# Autodesk Inventor assembly: FumeBOT
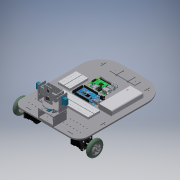
[picture p0: Inventor's stored thumbnail of the model, 180x180]
Saved by Autodesk Inventor 2018 (Build 220112000, 112)
## iProperties
Created: 2018-05-02
Part Number: FumeBOT
Document SubType Name: Assembly
Designer: Ajith Thomas
Author: Ajith Thomas
## Documents named in this file (11)
- C:\Users\Ajith Thomas\Dropbox\Gas_Sensing_Robot\FumeBot-Design\FumeBOT - with pan and tilt.iam
- C:\Users\Ajith Thomas\Dropbox\Gas_Sensing_Robot\FumeBot-Design\Base.ipt
- C:\Users\Ajith Thomas\Dropbox\Gas_Sensing_Robot\FumeBot-Design\Sensors and Boards\Raspberry Pi 3B.ipt
- C:\Users\Ajith Thomas\Dropbox\Gas_Sensing_Robot\FumeBot-Design\Sensors and Boards\Arduino MEGA 2560 R3\Arduino MEGA 2560 R3.iam
- C:\Users\Ajith Thomas\Dropbox\Gas_Sensing_Robot\FumeBot-Design\Large Bread Board.ipt
- C:\Users\Ajith Thomas\Dropbox\Gas_Sensing_Robot\FumeBot-Design\Small Bread Board.ipt
- C:\Users\Ajith Thomas\Dropbox\Gas_Sensing_Robot\FumeBot-Design\Battery.ipt
- C:\Users\Ajith Thomas\Dropbox\Gas_Sensing_Robot\FumeBot-Design\Stepper with bracket.iam
- C:\Users\Ajith Thomas\Dropbox\Gas_Sensing_Robot\FumeBot-Design\Wheel height spacers.ipt
- C:\Users\Ajith Thomas\Dropbox\Gas_Sensing_Robot\FumeBot-Design\Mecanum with supports.iam
- C:\Users\Ajith Thomas\Dropbox\Gas_Sensing_Robot\FumeBot-Design\Pan and tilt assembly\Camera pan and tilt assembly.iam
## Components (12 placed, 10 different names)
1. Base:1 — Mate:1, Mate:2, Flush:1, Flush:2, Flush:3, Flush:4, Mate:4, Mate:5, Mate:6, Flush:6, Flush:7, Mate:7, Mate:8, Mate:9, Mate:10, Mate:11, Mate:12, Flush:8, Mate:13
2. Raspberry Pi 3B:1 — Mate:10
3. Arduino MEGA 2560 R3:1 [sub-assembly] — Mate:9
4. Large Bread Board:1 — Mate:8
5. Small Bread Board:1 — Mate:11
6. Battery:1 — Mate:7
7. Stepper with bracket:1 [sub-assembly] — Mate:1, Flush:1, Flush:3, Flush:5
8. Stepper with bracket:2 [sub-assembly] — Mate:2, Flush:2, Flush:4, Mate:3
9. Wheel height spacers:1 — Flush:5
10. Wheel height spacers:2 — Mate:3, Mate:4, Mate:5
11. Mecanum with supports:1 [sub-assembly] — Mate:6, Flush:6, Flush:7
12. Camera pan and tilt assembly:1 [sub-assembly] — Mate:12, Flush:8, Mate:13
## Relationships (21: Mate 13, Flush 8)
- Mate:1 (6 mm): Base:1 ↔ Stepper with bracket:1
- Mate:2 (6 mm): Base:1 ↔ Stepper with bracket:2
- Flush:1 (20 mm): Base:1 ↔ Stepper with bracket:1
- Flush:2 (20 mm): Base:1 ↔ Stepper with bracket:2
- Flush:3 (30 mm): Base:1 ↔ Stepper with bracket:1
- Flush:4 (30 mm): Base:1 ↔ Stepper with bracket:2
- Flush:5: Stepper with bracket:1 ↔ Wheel height spacers:1
- Mate:3: Stepper with bracket:2 ↔ Wheel height spacers:2
- Mate:4: Base:1 ↔ Wheel height spacers:2
- Mate:5: Base:1 ↔ Wheel height spacers:2
- Mate:6: Base:1 ↔ Mecanum with supports:1
- Flush:6 (23 mm): Base:1 ↔ Mecanum with supports:1
- Flush:7 (121.1 mm): Base:1 ↔ Mecanum with supports:1
- Mate:7: Base:1 ↔ Battery:1
- Mate:8: Base:1 ↔ Large Bread Board:1
- Mate:9: Base:1 ↔ Arduino MEGA 2560 R3:1
- Mate:10: Base:1 ↔ Raspberry Pi 3B:1
- Mate:11: Base:1 ↔ Small Bread Board:1
- Mate:12: Base:1 ↔ Camera pan and tilt assembly:1
- Flush:8: Base:1 ↔ Camera pan and tilt assembly:1
- Mate:13: Base:1 ↔ Camera pan and tilt assembly:1
